# Autodesk Inventor assembly: RORPOS20-L30_MIR_MIR_MIR1
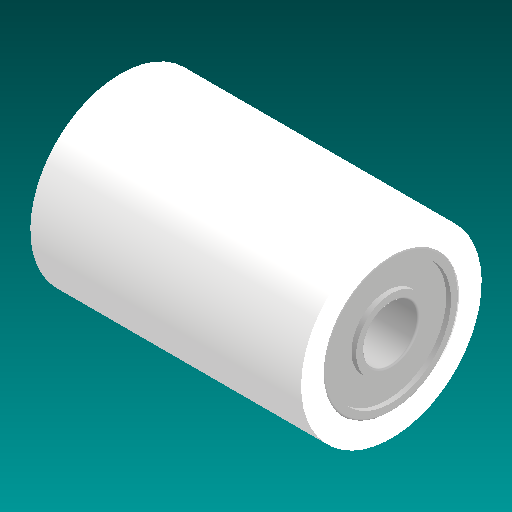
[picture p0: Inventor's stored thumbnail of the model, 512x512]
Saved by Autodesk Inventor 2020 (Build 240168000, 168)
## iProperties
Category: PARTsolutions
Company: MISUMI
Created: 2022-11-16
Part Number: RORPOS20-L30_MIR_MIR_MIR1
Catalog Web Link: www.cadenas.de
Description: RORPOS, RORPHS, RORPES, RORPJS, RORPSS, RORPQS, RORMCS-Plastic Roller -Milled/Straight-
Vendor: MISUMI
Document SubType Name: Assembly
Designer: kanazawakotaro
Manufacturer: MISUMI
Mass: 7.38247 g
Surface Area: 48.2474 cm^2
Volume: 7.38247 cm^3
Density: 1 g/cm^3
Title: RORPOS20-L30
Author: Cadenas PARTsolutions
Comments: Plastic Roller -Milled/Straight-
PSOL_IDENT_0: {$CADENAS_DATA/23d-libs/misumi/metric/53_rollers/rorpes_asmtab.prj},228 {VTYP=3D},{STYP=ASSTAB},{NB=
PSOL_IDENT_1: RORPOS20-L30},{LINA=RORPOS20-L30},{NN=RORPOS, RORPHS, RORPES, RORPJS, RORPSS, RORPQS, RORMCS},{DATE=
PSOL_IDENT_2: 30.06.2021 13:26:50},{GEOMDATE=18.05.2012},{VERSION=},{LINEID=10},{WBVAR=MAT,MATB,L},{WBNUMERIC=L}
PSOL_IDENT_3: {NB=RORPOS20-L30},{LINA=RORPOS20-L30},{KT=DUMMY},{PN=RORPOS20-L30},{TYPE=RORPOS},{MAT=1},{ALT1=},{MA
PSOL_IDENT_4: TB=S},{MATBALG= 'S', 'Steel', 'SS', 'Stainless Steel' },{MATB1=Steel},{MATB2=52100 Bearing Steel},{N
PSOL_IDENT_5: O=20},{NOM=20},{L=30},{L0=[15-100/1]},{BU=B696ZZx2},{BUN=696ZZ},{D=20},{D1=15},{DD=6},{B=5},{DDHH=10
PSOL_IDENT_6: },{PPATH=rorpos_asmtpl.prj}
NB: RORPOS20-L30
NN: RORPOS, RORPHS, RORPES, RORPJS, RORPSS, RORPQS, RORMCS
NT: Plastic Roller -Milled/Straight-
NBSYN: $PN.
LINA: RORPOS20-L30
CATALOG: Misumi
PN: RORPOS20-L30
MAT: Polyacetal
MATB: Steel
NO: 20
L: 30
BU: B696ZZx2
D: 20
D1: 15
DD: 6
B: 5
DDHH: 10
SUPPLIER: MISUMI
ARTICLENO: RORPOS20-L30
BOMINFO: RORPOS20-L30
CREATOR: CADENAS GmbH
## Documents named in this file (3)
- C:\Users\金澤航太郎\Documents\Inventor\kamuy2\Parts\RORPOS20-L30_Autodesk_Inventor_2020_20221117\AIS2020\RORPOS20-L30_MIR_MIR_MIR1.iam
- C:\Users\金澤航太郎\Documents\Inventor\kamuy2\Parts\RORPOS20-L30_Autodesk_Inventor_2020_20221117\AIS2020\RORPOS20-L30_1_MIR_MIR_MIR1.ipt
- C:\Users\金澤航太郎\Documents\Inventor\kamuy2\Parts\RORPOS20-L30_Autodesk_Inventor_2020_20221117\AIS2020\B696ZZ_MIR_MIR_MIR1.ipt
## Components (3 placed, 2 different names)
1. RORPOS20-L30_1_MIR_MIR_MIR1:1 — body_to_B_L__Z@1 <-> to_housing_Z@2, body_to_B_R__Z@1 <-> to_housing_Z@3
2. B696ZZ_MIR_MIR_MIR1:1 — body_to_B_L__Z@1 <-> to_housing_Z@2
3. B696ZZ_MIR_MIR_MIR1:2 — body_to_B_R__Z@1 <-> to_housing_Z@3
## Relationships (2: Mate 2)
- body_to_B_L__Z@1 <-> to_housing_Z@2 [Mate]: RORPOS20-L30_1_MIR_MIR_MIR1:1 ↔ B696ZZ_MIR_MIR_MIR1:1
- body_to_B_R__Z@1 <-> to_housing_Z@3 [Mate]: RORPOS20-L30_1_MIR_MIR_MIR1:1 ↔ B696ZZ_MIR_MIR_MIR1:2
